# Autodesk Inventor assembly: usp
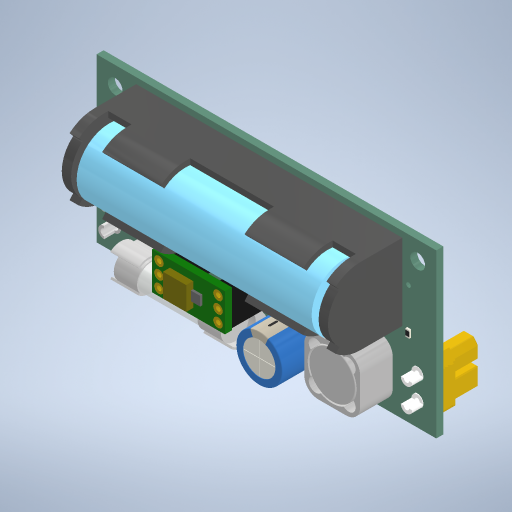
[picture p0: Inventor's stored thumbnail of the model, 512x512]
Saved by Autodesk Inventor 2024.1 (Build 281209000, 209)
## iProperties
Company: Kicad
Created: 2025-04-22
Part Number: usp
Description: KiCad electronic assembly
Document SubType Name: Assembly
Designer: hibik
Authority: Unknown
Sending System: KiCad to STEP converter
Preprocessor: Open CASCADE STEP processor 7.8
Title: power_assy.step
Author: Pcbnew
## Documents named in this file (17)
- C:\Users\hibik\Documents\Robomech\RESCUE\ORCA\hard\board\power_model\usp.iam
- C:\Users\hibik\Documents\Robomech\RESCUE\ORCA\hard\board\power_assy\C_0603_1608Metric.ipt
- C:\Users\hibik\Documents\Robomech\RESCUE\ORCA\hard\board\power_assy\smd_power_inductor.ipt
- C:\Users\hibik\Documents\Robomech\RESCUE\ORCA\hard\board\power_assy\TPS61230A.ipt
- C:\Users\hibik\Documents\Robomech\RESCUE\ORCA\hard\board\power_assy\R_0603_1608Metric.ipt
- C:\Users\hibik\Documents\Robomech\RESCUE\ORCA\hard\board\power_assy\AA_battery_set.iam
- C:\Users\hibik\Documents\Robomech\RESCUE\ORCA\hard\board\power_assy\LED_0603_1608Metric.ipt
- C:\Users\hibik\Documents\Robomech\RESCUE\ORCA\hard\board\power_assy\fuse.iam
- C:\Users\hibik\Documents\Robomech\RESCUE\ORCA\hard\board\power_assy\CP_Radial_D10.0mm_P5.00mm.ipt
- C:\Users\hibik\Documents\Robomech\RESCUE\ORCA\hard\board\power_assy\C_0805_2012Metric.ipt
- C:\Users\hibik\Documents\Robomech\RESCUE\ORCA\hard\board\power_assy\C_1206_3216Metric.ipt
- C:\Users\hibik\Documents\Robomech\RESCUE\ORCA\hard\board\power_assy\HTSOP-8-1EP_3.9x4.9mm_P1.27mm_EP2.4x3.2mm.ipt
- C:\Users\hibik\Documents\Robomech\RESCUE\ORCA\hard\board\power_assy\TSSOP-8_4.4x3mm_P0.65mm.ipt
- C:\Users\hibik\Documents\Robomech\RESCUE\ORCA\hard\board\power_assy\TSOT-23-6.ipt
- C:\Users\hibik\Documents\Robomech\RESCUE\ORCA\hard\board\power_assy\ORCA_power_board_PCB.ipt
- C:\Users\hibik\Documents\Robomech\RESCUE\ORCA\hard\board\power_assy\xt30_female.ipt
- C:\Users\hibik\Documents\Robomech\RESCUE\ORCA\hard\board\power_assy\xt30_male.ipt
## Components (47 placed, 47 different names)
1. 2
2. 3
3. 4
4. 10 [sub-assembly]
5. 14
6. 15
7. 16
8. 23
9. 27
10. 29
11. 33
12. 34
13. 35 [sub-assembly]
14. 36
15. 37
16. 38
17. 40
18. 41
19. 42
20. 47
21. 49
22. 50
23. 51
24. 52
25. 53
26. 54
27. 58
28. 60
29. 62
30. 63
31. 64
32. 66
33. 69
34. 71
35. 73
36. 76
37. 78
38. 87
39. 92
40. 93
41. 94
42. 99
43. 100
44. 104
45. 112 — 挿入:1, 挿入:2, 角度:1, 角度:2
46. xt30_female:1 — 挿入:2, 角度:1
47. xt30_male:1 — 挿入:1, 角度:2
## Relationships (4: Insert 2, Angle 2)
- 挿入:1 [Insert]: 112 ↔ xt30_male:1
- 挿入:2 [Insert]: 112 ↔ xt30_female:1
- 角度:1 [Angle] (0 deg): 112 ↔ xt30_female:1
- 角度:2 [Angle] (0 deg): 112 ↔ xt30_male:1
